# Autodesk Inventor assembly: CAD_Cubesat_3U
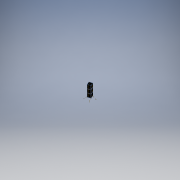
[picture p0: Inventor's stored thumbnail of the model, 180x180]
Saved by Autodesk Inventor 2017 (Build 210142000, 142)
## iProperties
Created: 2016-03-16
Part Number: CAD_Cubesat_3U
Document SubType Name: Assembly
Designer: Cosmonauta
Author: Cosmonauta
## Documents named in this file (12)
- C:\Users\Cosmonauta\ownCloud\Aurora\Proyectos\SUCHAI_2-3\Subsistemas\MEC\CAD_Cubesat3U\CAD_Cubesat_3U.iam
- C:\Users\Cosmonauta\ownCloud\Aurora\Proyectos\SUCHAI_2-3\Subsistemas\MEC\CAD_Cubesat3U\Structure\CAD\ISIS 3U Cubesat Structure.iam
- C:\Users\Cosmonauta\ownCloud\Aurora\Proyectos\SUCHAI_2-3\Subsistemas\MEC\CAD_Cubesat3U\NanoDock_OBC_TRX\Dock_OBC_TRX.iam
- C:\Users\Cosmonauta\ownCloud\Aurora\Proyectos\SUCHAI_2-3\Subsistemas\MEC\CAD_Cubesat3U\Nanopower_P110\CAD\p110-cad\A\P110UA.iam
- C:\Users\Cosmonauta\ownCloud\Aurora\Proyectos\SUCHAI_2-3\Subsistemas\MEC\CAD_Cubesat3U\Nanopower_P110\CAD\p110-cad\B\P110UB.iam
- C:\Users\Cosmonauta\ownCloud\Aurora\Proyectos\SUCHAI_2-3\Subsistemas\MEC\CAD_Cubesat3U\Nanopower_P110\CAD\p110-cad\C\P110UC.iam
- C:\Users\Cosmonauta\ownCloud\Aurora\Proyectos\SUCHAI_2-3\Subsistemas\MEC\CAD_Cubesat3U\Nanopower_plus_BP4\Nanopower_plus_BP4.iam
- C:\Users\Cosmonauta\ownCloud\Aurora\Proyectos\SUCHAI_2-3\Subsistemas\MEC\CAD_Cubesat3U\Nanopower_P110\CAD\p110-cad\C\nanocom-ant430-deployed.iam
- C:\Users\Cosmonauta\ownCloud\Aurora\Proyectos\SUCHAI_2-3\Subsistemas\MEC\CAD_Cubesat3U\Insterstage_panels\CAD\GOMX-Interstage-B.ipt
- C:\Users\Cosmonauta\ownCloud\Aurora\Proyectos\SUCHAI_2-3\Subsistemas\MEC\CAD_Cubesat3U\Insterstage_panels\CAD\GOMX-Interstage-FPP.iam
- C:\Users\Cosmonauta\ownCloud\Aurora\Proyectos\SUCHAI_2-3\Subsistemas\MEC\CAD_Cubesat3U\Insterstage_panels\CAD\GOMX-Interstage-A.ipt
- C:\Users\Cosmonauta\ownCloud\Aurora\Proyectos\SUCHAI_2-3\Subsistemas\MEC\CAD_Cubesat3U\NanoDock\CAD\Motherboard.iam
## Components (29 placed, 11 different names)
1. ISIS 3U Cubesat Structure:1 [sub-assembly] — Mate:1, Mate:2, Mate:3, Mate:4, Mate:5, Mate:6, Mate:7, Mate:8, Mate:9, Mate:10, Mate:11, Mate:12, Mate:13, Mate:14, Mate:15, Mate:16, Mate:17, Mate:18, Mate:19, Mate:20, Mate:21, Mate:22, Mate:23, Mate:24, Mate:25, Mate:26, Mate:27, Mate:28, Mate:29, Mate:30, Mate:31, Mate:32, Mate:33, Mate:34, Mate:35, Mate:36, Mate:37, Mate:38, Mate:39, Mate:40, Mate:41, Mate:54, Mate:55, Mate:56, Mate:57, Mate:58, Mate:59, Mate:60, Mate:61, Mate:62, Mate:63, Mate:64, Mate:65, Mate:66, Mate:67, Mate:68, Mate:69, Mate:70, Mate:71, Mate:72, Mate:73, Mate:74, Mate:75, Mate:76, Mate:77, Mate:78, Mate:79, Mate:80
2. Dock_OBC_TRX:1 [sub-assembly] — Mate:1, Mate:2, Mate:45, Mate:46, Mate:47
3. P110UB:1 [sub-assembly] — Mate:3, Mate:4, Mate:5
4. P110UB:2 [sub-assembly] — Mate:12, Mate:13, Mate:14
5. P110UB:3 [sub-assembly] — Mate:18, Mate:19, Mate:20
6. P110UB:4 [sub-assembly] — Mate:15, Mate:16, Mate:17
7. P110UB:5 [sub-assembly] — Mate:9, Mate:10, Mate:11
8. P110UB:6 [sub-assembly] — Mate:6, Mate:7, Mate:8
9. P110UA:1 [sub-assembly] — Mate:21, Mate:22, Mate:23
10. P110UA:2 [sub-assembly] — Mate:27, Mate:28, Mate:29
11. P110UA:3 [sub-assembly] — Mate:24, Mate:25, Mate:26
12. P110UA:4 [sub-assembly] — Mate:36, Mate:37, Mate:38
13. P110UA:5 [sub-assembly] — Mate:33, Mate:34, Mate:35
14. P110UA:6 [sub-assembly] — Mate:30, Mate:31, Mate:32
15. P110UC:1 [sub-assembly] — Mate:39, Mate:40, Mate:41
16. Nanopower_plus_BP4:1 [sub-assembly] — Mate:45, Mate:46, Mate:47
17. nanocom-ant430-deployed:1 [sub-assembly]
18. P110UC:2 [sub-assembly]
19. GOMX-Interstage-B:1 — Mate:54, Mate:55, Mate:56
20. GOMX-Interstage-B:2 — Mate:57, Mate:58, Mate:59
21. GOMX-Interstage-B:3 — Mate:60, Mate:61, Mate:62
22. GOMX-Interstage-B:4 — Mate:63, Mate:64, Mate:65
23. GOMX-Interstage-FPP:1 [sub-assembly] — Mate:75, Mate:76, Mate:77
24. GOMX-Interstage-A:2 — Mate:69, Mate:70, Mate:71
25. GOMX-Interstage-A:3 — Mate:72, Mate:73, Mate:74
26. GOMX-Interstage-A:4 — Mate:66, Mate:67, Mate:68
27. Motherboard:1 [sub-assembly] — Mate:78, Mate:79, Mate:80, Mate:81, Mate:82, Mate:83
28. Motherboard:2 [sub-assembly] — Mate:81, Mate:82, Mate:83, Mate:84, Mate:85, Mate:86
29. Motherboard:3 [sub-assembly] — Mate:84, Mate:85, Mate:86
## Relationships (83: Mate 83)
- Mate:1: ISIS 3U Cubesat Structure:1 ↔ Dock_OBC_TRX:1
- Mate:2: ISIS 3U Cubesat Structure:1 ↔ Dock_OBC_TRX:1
- Mate:3: ISIS 3U Cubesat Structure:1 ↔ P110UB:1
- Mate:4: ISIS 3U Cubesat Structure:1 ↔ P110UB:1
- Mate:5: ISIS 3U Cubesat Structure:1 ↔ P110UB:1
- Mate:6: ISIS 3U Cubesat Structure:1 ↔ P110UB:6
- Mate:7: ISIS 3U Cubesat Structure:1 ↔ P110UB:6
- Mate:8: ISIS 3U Cubesat Structure:1 ↔ P110UB:6
- Mate:9: ISIS 3U Cubesat Structure:1 ↔ P110UB:5
- Mate:10: ISIS 3U Cubesat Structure:1 ↔ P110UB:5
- Mate:11: ISIS 3U Cubesat Structure:1 ↔ P110UB:5
- Mate:12: ISIS 3U Cubesat Structure:1 ↔ P110UB:2
- Mate:13: ISIS 3U Cubesat Structure:1 ↔ P110UB:2
- Mate:14: ISIS 3U Cubesat Structure:1 ↔ P110UB:2
- Mate:15: ISIS 3U Cubesat Structure:1 ↔ P110UB:4
- Mate:16: ISIS 3U Cubesat Structure:1 ↔ P110UB:4
- Mate:17: ISIS 3U Cubesat Structure:1 ↔ P110UB:4
- Mate:18: ISIS 3U Cubesat Structure:1 ↔ P110UB:3
- Mate:19: ISIS 3U Cubesat Structure:1 ↔ P110UB:3
- Mate:20: ISIS 3U Cubesat Structure:1 ↔ P110UB:3
- Mate:21: ISIS 3U Cubesat Structure:1 ↔ P110UA:1
- Mate:22: ISIS 3U Cubesat Structure:1 ↔ P110UA:1
- Mate:23: ISIS 3U Cubesat Structure:1 ↔ P110UA:1
- Mate:24: ISIS 3U Cubesat Structure:1 ↔ P110UA:3
- Mate:25: ISIS 3U Cubesat Structure:1 ↔ P110UA:3
- Mate:26: ISIS 3U Cubesat Structure:1 ↔ P110UA:3
- Mate:27: ISIS 3U Cubesat Structure:1 ↔ P110UA:2
- Mate:28: ISIS 3U Cubesat Structure:1 ↔ P110UA:2
- Mate:29: ISIS 3U Cubesat Structure:1 ↔ P110UA:2
- Mate:30: ISIS 3U Cubesat Structure:1 ↔ P110UA:6
- Mate:31: ISIS 3U Cubesat Structure:1 ↔ P110UA:6
- Mate:32: ISIS 3U Cubesat Structure:1 ↔ P110UA:6
- Mate:33: ISIS 3U Cubesat Structure:1 ↔ P110UA:5
- Mate:34: ISIS 3U Cubesat Structure:1 ↔ P110UA:5
- Mate:35: ISIS 3U Cubesat Structure:1 ↔ P110UA:5
- Mate:36: ISIS 3U Cubesat Structure:1 ↔ P110UA:4
- Mate:37: ISIS 3U Cubesat Structure:1 ↔ P110UA:4
- Mate:38: ISIS 3U Cubesat Structure:1 ↔ P110UA:4
- Mate:39: ISIS 3U Cubesat Structure:1 ↔ P110UC:1
- Mate:40: ISIS 3U Cubesat Structure:1 ↔ P110UC:1
- Mate:41: ISIS 3U Cubesat Structure:1 ↔ P110UC:1
- Mate:45 (15 mm): Dock_OBC_TRX:1 ↔ Nanopower_plus_BP4:1
- Mate:46: Dock_OBC_TRX:1 ↔ Nanopower_plus_BP4:1
- Mate:47: Dock_OBC_TRX:1 ↔ Nanopower_plus_BP4:1
- [Mate]: ISIS 3U Cubesat Structure:1 ↔ nanocom-ant430-deployed:1
- [Mate]: ISIS 3U Cubesat Structure:1 ↔ nanocom-ant430-deployed:1
- [Mate]: ISIS 3U Cubesat Structure:1 ↔ nanocom-ant430-deployed:1
- [Mate]: nanocom-ant430-deployed:1 ↔ P110UC:2
- [Mate]: nanocom-ant430-deployed:1 ↔ P110UC:2
- [Mate]: nanocom-ant430-deployed:1 ↔ P110UC:2
- Mate:54: ISIS 3U Cubesat Structure:1 ↔ GOMX-Interstage-B:1
- Mate:55: ISIS 3U Cubesat Structure:1 ↔ GOMX-Interstage-B:1
- Mate:56 (0.2 mm): ISIS 3U Cubesat Structure:1 ↔ GOMX-Interstage-B:1
- Mate:57: ISIS 3U Cubesat Structure:1 ↔ GOMX-Interstage-B:2
- Mate:58: ISIS 3U Cubesat Structure:1 ↔ GOMX-Interstage-B:2
- Mate:59 (0.2 mm): ISIS 3U Cubesat Structure:1 ↔ GOMX-Interstage-B:2
- Mate:60: ISIS 3U Cubesat Structure:1 ↔ GOMX-Interstage-B:3
- Mate:61: ISIS 3U Cubesat Structure:1 ↔ GOMX-Interstage-B:3
- Mate:62 (0.2 mm): ISIS 3U Cubesat Structure:1 ↔ GOMX-Interstage-B:3
- Mate:63: ISIS 3U Cubesat Structure:1 ↔ GOMX-Interstage-B:4
- Mate:64: ISIS 3U Cubesat Structure:1 ↔ GOMX-Interstage-B:4
- Mate:65 (0.2 mm): ISIS 3U Cubesat Structure:1 ↔ GOMX-Interstage-B:4
- Mate:66: ISIS 3U Cubesat Structure:1 ↔ GOMX-Interstage-A:4
- Mate:67: ISIS 3U Cubesat Structure:1 ↔ GOMX-Interstage-A:4
- Mate:68 (0.2 mm): ISIS 3U Cubesat Structure:1 ↔ GOMX-Interstage-A:4
- Mate:69: ISIS 3U Cubesat Structure:1 ↔ GOMX-Interstage-A:2
- Mate:70: ISIS 3U Cubesat Structure:1 ↔ GOMX-Interstage-A:2
- Mate:71 (0.2 mm): ISIS 3U Cubesat Structure:1 ↔ GOMX-Interstage-A:2
- Mate:72: ISIS 3U Cubesat Structure:1 ↔ GOMX-Interstage-A:3
- Mate:73: ISIS 3U Cubesat Structure:1 ↔ GOMX-Interstage-A:3
- Mate:74 (0.2 mm): ISIS 3U Cubesat Structure:1 ↔ GOMX-Interstage-A:3
- Mate:75: ISIS 3U Cubesat Structure:1 ↔ GOMX-Interstage-FPP:1
- Mate:76: ISIS 3U Cubesat Structure:1 ↔ GOMX-Interstage-FPP:1
- Mate:77 (0.2 mm): ISIS 3U Cubesat Structure:1 ↔ GOMX-Interstage-FPP:1
- Mate:78: ISIS 3U Cubesat Structure:1 ↔ Motherboard:1
- Mate:79: ISIS 3U Cubesat Structure:1 ↔ Motherboard:1
- Mate:80 (0.1 mm): ISIS 3U Cubesat Structure:1 ↔ Motherboard:1
- Mate:81 (30 mm): Motherboard:1 ↔ Motherboard:2
- Mate:82: Motherboard:1 ↔ Motherboard:2
- Mate:83: Motherboard:1 ↔ Motherboard:2
- Mate:84 (15 mm): Motherboard:2 ↔ Motherboard:3
- Mate:85: Motherboard:2 ↔ Motherboard:3
- Mate:86: Motherboard:2 ↔ Motherboard:3
